# Autodesk Inventor assembly: 装配-输肉通道
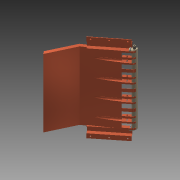
[picture p0: Inventor's stored thumbnail of the model, 180x180]
Saved by Autodesk Inventor 2015 (Build 190159000, 159)
## iProperties
Created: 2017-05-24
Part Number: 装配-输肉通道
Document SubType Name: Assembly
Designer: Administrator
Author: Administrator
## Documents named in this file (5)
- C:\Users\Administrator\Desktop\毕设改终\装配-输肉通道.iam
- C:\Users\Administrator\Desktop\毕设改终\分离水箱.ipt
- C:\Users\Administrator\Desktop\毕设改终\分离水箱固定螺帽.ipt
- C:\Users\Administrator\Desktop\毕设改终\分离水箱固定螺丝.ipt
- C:\Users\Administrator\Desktop\毕设改终\输肉通道.ipt
## Components (10 placed, 4 different names)
1. 分离水箱:1 — 插入:1, 插入:2, 配合:1
2. 输肉通道:1 — 插入:1, 插入:2, 插入:3
3. 分离水箱固定螺帽:1 — 插入:3
4. 分离水箱固定螺丝:1 — 配合:1
5. 分离水箱固定螺帽:2
6. 分离水箱固定螺丝:2
7. 分离水箱固定螺帽:3
8. 分离水箱固定螺丝:3
9. 分离水箱固定螺帽:4
10. 分离水箱固定螺丝:4
## Component patterns: (2 elements), (2 elements, first: 分离水箱固定螺帽:1 + 分离水箱固定螺丝:1), 零部件阵列 1:2 (2 elements)
## Relationships (4: Insert 3, Mate 1)
- 插入:1 [Insert]: 分离水箱:1 ↔ 输肉通道:1
- 插入:2 [Insert]: 分离水箱:1 ↔ 输肉通道:1
- 配合:1 [Mate]: 分离水箱:1 ↔ 分离水箱固定螺丝:1
- 插入:3 [Insert]: 输肉通道:1 ↔ 分离水箱固定螺帽:1
